# Autodesk Inventor assembly: SensorAssembly
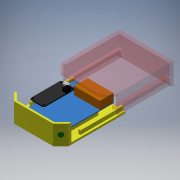
[picture p0: Inventor's stored thumbnail of the model, 180x180]
Saved by Autodesk Inventor 2018 (Build 220112000, 112)
## iProperties
Created: 2019-10-14
Part Number: SensorAssembly
Document SubType Name: Assembly
Designer: jklei
Author: jklei
## Documents named in this file (8)
- C:\Users\jklei\Desktop\Wildfire-Detector\CAD\SensorAssembly.iam
- C:\Users\jklei\Desktop\Wildfire-Detector\CAD\2829 Adafruit Feather Bluefruit 32u4.ipt
- C:\Users\jklei\Desktop\Wildfire-Detector\CAD\sensor.ipt
- C:\Users\jklei\Desktop\Wildfire-Detector\CAD\bottom-housing.ipt
- C:\Users\jklei\Desktop\Wildfire-Detector\CAD\top-slider.ipt
- C:\Users\jklei\Desktop\Wildfire-Detector\CAD\PCB.ipt
- C:\Users\jklei\Desktop\Wildfire-Detector\CAD\Battery.ipt
- C:\Users\jklei\Desktop\Wildfire-Detector\CAD\BoostConverter.ipt
## Components (8 placed, 7 different names)
1. 2829 Adafruit Feather Bluefruit 32u4:1 — Flush:3, Mate:18, Flush:4
2. sensor:1 — Insert:2
3. sensor:2 — Insert:1
4. bottom-housing:1 — Flush:1, Mate:6, Insert:1, Insert:2, Mate:9, Mate:10, Mate:11, Mate:16, Mate:17
5. top-slider:1 — Flush:1, Mate:6
6. PCB:1 — Flush:3, Mate:9, Mate:10, Mate:12, Mate:18, Flush:4, Flush:5, Mate:19, Flush:6
7. Battery:1 — Mate:11, Mate:12, Mate:16, Mate:17
8. BoostConverter:1 — Flush:5, Mate:19, Flush:6
## Relationships (16: Mate 9, Flush 5, Insert 2)
- Flush:1: bottom-housing:1 ↔ top-slider:1
- Mate:6: bottom-housing:1 ↔ top-slider:1
- Insert:1: sensor:2 ↔ bottom-housing:1
- Insert:2: sensor:1 ↔ bottom-housing:1
- Flush:3 (23.175 mm): 2829 Adafruit Feather Bluefruit 32u4:1 ↔ PCB:1
- Mate:9 (6.985 mm): bottom-housing:1 ↔ PCB:1
- Mate:10 (5.08 mm): bottom-housing:1 ↔ PCB:1
- Mate:11: bottom-housing:1 ↔ Battery:1
- Mate:12: PCB:1 ↔ Battery:1
- Mate:16: bottom-housing:1 ↔ Battery:1
- Mate:17: bottom-housing:1 ↔ Battery:1
- Mate:18 (9.525 mm): 2829 Adafruit Feather Bluefruit 32u4:1 ↔ PCB:1
- Flush:4: 2829 Adafruit Feather Bluefruit 32u4:1 ↔ PCB:1
- Flush:5: PCB:1 ↔ BoostConverter:1
- Mate:19: PCB:1 ↔ BoostConverter:1
- Flush:6: PCB:1 ↔ BoostConverter:1
